# Autodesk Inventor assembly: Camera.assembly
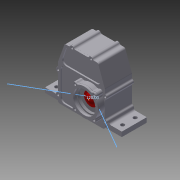
[picture p0: Inventor's stored thumbnail of the model, 180x180]
Saved by Autodesk Inventor 2011 (Build 150239000, 239)
## iProperties
Created: 2011-03-21
Part Number: Camera.assembly
Document SubType Name: Assembly
Designer: Rob
Mass: 331.167 g
Surface Area: 902.13 cm^2
Volume: 173.288 cm^3
Density: 1.91108 g/cm^3
Author: Rob
## Documents named in this file (7)
- C:\Users\M. Woods III\Desktop\design\Mechanical Drawings\camera.iam
- C:\Users\M. Woods III\Desktop\design\Mechanical Drawings\camera_Back.ipt
- C:\Users\M. Woods III\Desktop\design\Mechanical Drawings\Camera.ipt
- C:\Users\M. Woods III\Desktop\design\Mechanical Drawings\camera_glass.ipt
- C:\Users\M. Woods III\Desktop\design\Mechanical Drawings\camera_front.ipt
- C:\Users\M. Woods III\Desktop\design\Mechanical Drawings\camera_glassmount.ipt
- C:\Users\M. Woods III\Desktop\design\Mechanical Drawings\camera_silicon.ipt
## Components (6 placed, 6 different names)
1. camera_Back:1 — Flush:1, Flush:2, Mate:4, Mate:5, Mate:8, Mate:9, Mate:10
2. Camera:1 — Mate:4, Mate:5, Mate:11
3. camera_glass:1 — Mate:6, Mate:7
4. camera_front:1 — Flush:1, Flush:2, Mate:1, Mate:2, Mate:3, Mate:6, Mate:7
5. camera_glassmount:1 — Mate:1, Mate:2, Mate:3
6. camera_silicon:1 — Mate:8, Mate:9, Mate:10, Mate:11
## Relationships (13: Mate 11, Flush 2)
- Flush:1: camera_Back:1 ↔ camera_front:1
- Flush:2: camera_Back:1 ↔ camera_front:1
- Mate:1: camera_front:1 ↔ camera_glassmount:1
- Mate:2: camera_front:1 ↔ camera_glassmount:1
- Mate:3: camera_front:1 ↔ camera_glassmount:1
- Mate:4 (2 mm): camera_Back:1 ↔ Camera:1
- Mate:5 (2 mm): camera_Back:1 ↔ Camera:1
- Mate:6: camera_glass:1 ↔ camera_front:1
- Mate:7: camera_glass:1 ↔ camera_front:1
- Mate:8: camera_Back:1 ↔ camera_silicon:1
- Mate:9: camera_Back:1 ↔ camera_silicon:1
- Mate:10: camera_Back:1 ↔ camera_silicon:1
- Mate:11: Camera:1 ↔ camera_silicon:1
